# Autodesk Inventor assembly: Backpack
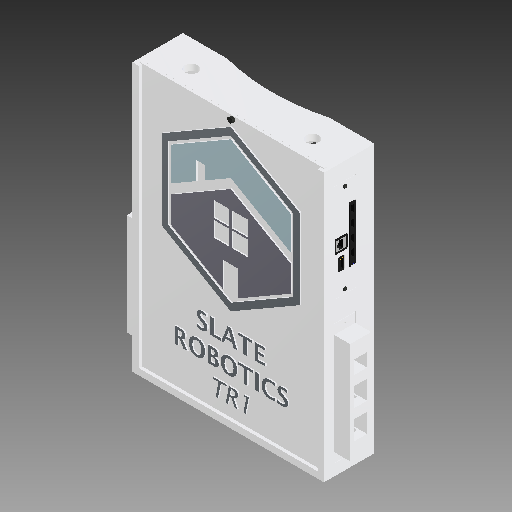
[picture p0: Inventor's stored thumbnail of the model, 512x512]
Saved by Autodesk Inventor 2017 (Build 210142000, 142)
## iProperties
Created: 2017-09-05
Part Number: Backpack
Document SubType Name: Assembly
Designer: Zach
Author: Zach
## Documents named in this file (18)
- C:\Users\Dell\Documents\GitHub\tr1\src\Body\Chest Assembly\Backpack Assembly\Backpack.iam
- C:\Users\Dell\Documents\GitHub\tr1\src\Body\Chest Assembly\Backpack Assembly\BP001b.ipt
- C:\Users\Dell\Documents\GitHub\tr1\src\Body\Chest Assembly\Backpack Assembly\BP002b.ipt
- C:\Users\Dell\Documents\GitHub\tr1\src\Body\Chest Assembly\Backpack Assembly\BP003.ipt
- C:\Users\Dell\Documents\GitHub\tr1\src\Body\Chest Assembly\Backpack Assembly\BP005.ipt
- C:\Users\Dell\Documents\GitHub\tr1\src\Body\Chest Assembly\Backpack Assembly\BP006.ipt
- C:\Users\Dell\Documents\GitHub\tr1\lib\Terminal Block 4\Клемная колодка ТВ-2504L 600V-25A\Клемная колодка ТВ-2504L 600V-25A.iam
- C:\Users\Dell\Documents\GitHub\tr1\lib\Arduino Mega 2560\Arduino Mega 2560.ipt
- C:\Users\Dell\Documents\GitHub\tr1\lib\L298n Driver\l298n.ipt
- C:\Users\Dell\Documents\GitHub\tr1\lib\Content Center Files\R2017\en-US\ISO 7045  H\ISO 7045 - M3 x 12 - 4.8 - H - ISO.ipt
- C:\Users\Dell\Documents\GitHub\tr1\lib\Content Center Files\R2017\en-US\ISO 4018\ISO 4018 - M5 x 25.ipt
- C:\Users\Dell\Documents\GitHub\tr1\src\Body\Chest Assembly\Backpack Assembly\USB Hub.ipt
- C:\Users\Dell\Documents\GitHub\tr1\src\Body\Chest Assembly\Backpack Assembly\HDMI Port.ipt
- C:\Users\Dell\Documents\GitHub\tr1\src\Body\Chest Assembly\Backpack Assembly\Ethernet Port.ipt
- C:\Users\Dell\Documents\GitHub\tr1\lib\Content Center Files\R2017\en-US\ISO 4035(2)\ISO 4035 - M3 - ISO.ipt
- C:\Users\Dell\Documents\GitHub\tr1\src\Body\Chest Assembly\Backpack Assembly\BP011.ipt
- C:\Users\Dell\Documents\GitHub\tr1\src\Body\Chest Assembly\Backpack Assembly\BP012.ipt
- C:\Users\Dell\Documents\GitHub\tr1\src\Body\Chest Assembly\Backpack Assembly\BP013.ipt
## Components (84 placed, 17 different names)
1. BP001b:1 — Mate:8, Mate:9, Mate:11, Mate:13, Mate:15, Mate:19, Mate:20, Mate:21, Mate:22, Mate:23, Flush:1, Mate:26, Mate:36, Mate:37, Mate:38, Mate:39, Mate:133, Mate:134, Mate:137, Mate:138, Mate:160, Mate:162, Mate:163, Mate:176, Mate:177, Mate:178, Mate:179, Mate:180, Mate:181, Mate:182, Mate:183, Mate:184, Mate:185, Mate:186, Mate:187, Mate:188, Mate:189, Mate:190, Mate:191, Mate:310, Mate:312, Mate:314, Mate:316, Mate:317, Mate:318, Mate:319, Mate:326, Mate:327, Mate:328, Mate:330, Mate:331, Mate:332, Mate:334, Mate:335, Mate:336, Mate:337, Mate:338, Mate:339, Mate:340, Mate:341, Mate:342, Mate:343, Mate:344, Mate:345, Mate:346, Mate:347, Mate:348, Mate:349, Mate:350, Mate:351
2. BP002b:1 — Mate:317, Mate:318, Mate:319, Mate:333
3. BP003:1 — Mate:15, Mate:36, Mate:37, Mate:65, Mate:66, Mate:67, Mate:68, Mate:69, Mate:70, Mate:135, Mate:136, Mate:232, Mate:233, Mate:234, Mate:235, Mate:236, Mate:237, Mate:238, Mate:239, Mate:240, Mate:241, Mate:242, Mate:243
4. BP003:2 — Mate:19, Mate:38, Mate:39, Mate:59, Mate:60, Mate:61, Mate:62, Mate:63, Mate:64, Mate:139, Mate:140, Mate:208, Mate:209, Mate:210, Mate:211, Mate:212, Mate:213, Mate:214, Mate:215, Mate:216, Mate:217, Mate:218, Mate:219
5. BP005:1 — Mate:8, Mate:9, Mate:20, Mate:172, Mate:173, Mate:174, Mate:175, Mate:307, Mate:308
6. BP006:1 — Mate:11, Mate:13, Mate:21, Mate:168, Mate:169, Mate:170, Mate:171, Flush:6, Mate:282, Mate:283, Flush:7, Mate:284, Mate:285, Flush:8, Mate:286
7. BP011:1 — Mate:342, Mate:343, Mate:344
8. BP012:1 — Mate:345, Mate:346, Mate:347
9. BP013:1 — Mate:348, Mate:349, Mate:351
10. Клемная колодка ТВ-2504L 600V-25A:1 [sub-assembly] — Mate:26, Mate:337, Mate:338
11. Клемная колодка ТВ-2504L 600V-25A:2 [sub-assembly] — Mate:339, Mate:340, Mate:341
12. Клемная колодка ТВ-2504L 600V-25A:3 [sub-assembly] — Mate:334, Mate:335, Mate:336
13. Arduino Mega 2560:1 — Mate:96, Mate:116, Mate:117, Mate:118, Mate:119, Mate:120, Mate:327, Mate:328, Mate:329
14. Arduino Mega 2560:2 — Mate:127, Mate:128, Mate:129, Mate:130, Mate:131, Mate:132, Mate:326, Mate:330, Mate:331
15. l298n:1 — Mate:59, Mate:60, Flush:3, Mate:228, Mate:229, Mate:230, Mate:231
16. l298n:2 — Mate:62, Mate:63, Flush:2, Flush:3, Mate:224, Mate:225, Mate:226, Mate:227
17. l298n:3 — Mate:61, Mate:64, Flush:2, Mate:220, Mate:221, Mate:222, Mate:223
18. l298n:4 — Mate:67, Mate:70, Flush:4, Flush:5, Mate:248, Mate:249, Mate:250, Mate:251
19. l298n:5 — Mate:68, Mate:69, Flush:5, Mate:252, Mate:253, Mate:254, Mate:255
20. l298n:6 — Mate:65, Mate:66, Flush:4, Mate:244, Mate:245, Mate:246, Mate:247
21. USB Hub:1 — Flush:6, Mate:286, Mate:350
22. HDMI Port:1 — Mate:282, Mate:283, Flush:7
23. Ethernet Port:1 — Mate:284, Mate:285, Flush:8
24. ISO 7045 H M3 x 12 - 4.8 - H:1 — Mate:96, Mate:329
25. ISO 7045 H M3 x 12 - 4.8 - H:2 — Mate:117
26. ISO 7045 H M3 x 12 - 4.8 - H:3 — Mate:119
27. ISO 7045 H M3 x 12 - 4.8 - H:4 — Mate:120
28. ISO 7045 H M3 x 12 - 4.8 - H:5 — Mate:118
29. ISO 7045 H M3 x 12 - 4.8 - H:6 — Mate:116
30. ISO 7045 H M3 x 12 - 4.8 - H:7 — Mate:128
31. ISO 7045 H M3 x 12 - 4.8 - H:8 — Mate:131
32. ISO 7045 H M3 x 12 - 4.8 - H:9 — Mate:132
33. ISO 7045 H M3 x 12 - 4.8 - H:10 — Mate:129
34. ISO 7045 H M3 x 12 - 4.8 - H:11 — Mate:130
35. ISO 7045 H M3 x 12 - 4.8 - H:12 — Mate:127
36. ISO 7045 H M3 x 12 - 4.8 - H:13 — Mate:133, Mate:136
37. ISO 7045 H M3 x 12 - 4.8 - H:14 — Mate:134, Mate:135
38. ISO 7045 H M3 x 12 - 4.8 - H:15 — Mate:137, Mate:139
39. ISO 7045 H M3 x 12 - 4.8 - H:16 — Mate:138, Mate:140
40. ISO 7045 H M3 x 12 - 4.8 - H:27 — Mate:160
41. ISO 7045 H M3 x 12 - 4.8 - H:28 — Mate:163
42. ISO 7045 H M3 x 12 - 4.8 - H:30 — Mate:162
43. ISO 7045 H M3 x 12 - 4.8 - H:31 — Mate:169, Mate:170, Mate:313
44. ISO 7045 H M3 x 12 - 4.8 - H:32 — Mate:168, Mate:171, Mate:315
45. ISO 7045 H M3 x 12 - 4.8 - H:33 — Mate:172, Mate:173, Mate:309
46. ISO 7045 H M3 x 12 - 4.8 - H:34 — Mate:174, Mate:175
47. ISO 4018 M5 x 25:5 — Mate:179, Mate:190
48. ISO 4018 M5 x 25:6 — Mate:181, Mate:186
49. ISO 4018 M5 x 25:7 — Mate:182, Mate:187
50. ISO 4018 M5 x 25:8 — Mate:180, Mate:189
51. ISO 4018 M5 x 25:9 — Mate:177, Mate:191
52. ISO 4018 M5 x 25:10 — Mate:176, Mate:184
53. ISO 4018 M5 x 25:11 — Mate:178, Mate:185
54. ISO 4018 M5 x 25:12 — Mate:183, Mate:188
55. ISO 7045 H M3 x 12 - 4.8 - H:35 — Mate:219, Mate:230
56. ISO 7045 H M3 x 12 - 4.8 - H:36 — Mate:218, Mate:229
57. ISO 7045 H M3 x 12 - 4.8 - H:37 — Mate:217, Mate:228
58. ISO 7045 H M3 x 12 - 4.8 - H:38 — Mate:215, Mate:225
59. ISO 7045 H M3 x 12 - 4.8 - H:39 — Mate:216, Mate:231
60. ISO 7045 H M3 x 12 - 4.8 - H:40 — Mate:214, Mate:224
61. ISO 7045 H M3 x 12 - 4.8 - H:41 — Mate:213, Mate:226
62. ISO 7045 H M3 x 12 - 4.8 - H:42 — Mate:211, Mate:222
63. ISO 7045 H M3 x 12 - 4.8 - H:43 — Mate:210, Mate:223
64. ISO 7045 H M3 x 12 - 4.8 - H:44 — Mate:212, Mate:227
65. ISO 7045 H M3 x 12 - 4.8 - H:45 — Mate:209, Mate:220
66. ISO 7045 H M3 x 12 - 4.8 - H:46 — Mate:208, Mate:221
67. ISO 7045 H M3 x 12 - 4.8 - H:47 — Mate:238, Mate:248
68. ISO 7045 H M3 x 12 - 4.8 - H:48 — Mate:239, Mate:250
69. ISO 7045 H M3 x 12 - 4.8 - H:49 — Mate:243, Mate:254
70. ISO 7045 H M3 x 12 - 4.8 - H:50 — Mate:242, Mate:255
71. ISO 7045 H M3 x 12 - 4.8 - H:51 — Mate:232, Mate:245
72. ISO 7045 H M3 x 12 - 4.8 - H:52 — Mate:233, Mate:244
73. ISO 7045 H M3 x 12 - 4.8 - H:53 — Mate:235, Mate:246
74. ISO 7045 H M3 x 12 - 4.8 - H:54 — Mate:234, Mate:247
75. ISO 7045 H M3 x 12 - 4.8 - H:55 — Mate:236, Mate:249
76. ISO 7045 H M3 x 12 - 4.8 - H:56 — Mate:237, Mate:251
77. ISO 7045 H M3 x 12 - 4.8 - H:57 — Mate:240, Mate:253
78. ISO 7045 H M3 x 12 - 4.8 - H:58 — Mate:241, Mate:252
79. ISO 7045 H M3 x 12 - 4.8 - H:67 — Mate:307, Mate:308, Mate:311
80. ISO 4035 M3:1 — Mate:309, Mate:310
81. ISO 4035 M3:2 — Mate:311, Mate:312
82. ISO 4035 M3:3 — Mate:313, Mate:314
83. ISO 4035 M3:4 — Mate:315, Mate:316
84. ISO 4018 M5 x 25:13 — Mate:332, Mate:333
## Relationships (174: Mate 166, Flush 8)
- Mate:8: BP001b:1 ↔ BP005:1
- Mate:9: BP001b:1 ↔ BP005:1
- Mate:11: BP001b:1 ↔ BP006:1
- Mate:13: BP001b:1 ↔ BP006:1
- Mate:15: BP001b:1 ↔ BP003:1
- Mate:19: BP001b:1 ↔ BP003:2
- Mate:20: BP001b:1 ↔ BP005:1
- Mate:21: BP001b:1 ↔ BP006:1
- Mate:22: BP001b:1
- Mate:23: BP001b:1
- Flush:1 (200 mm): BP001b:1
- Mate:26: BP001b:1 ↔ Клемная колодка ТВ-2504L 600V-25A:1
- Mate:36: BP001b:1 ↔ BP003:1
- Mate:37: BP001b:1 ↔ BP003:1
- Mate:38: BP001b:1 ↔ BP003:2
- Mate:39: BP001b:1 ↔ BP003:2
- Mate:59: BP003:2 ↔ l298n:1
- Mate:60: BP003:2 ↔ l298n:1
- Mate:61: BP003:2 ↔ l298n:3
- Mate:62: BP003:2 ↔ l298n:2
- Mate:63: BP003:2 ↔ l298n:2
- Mate:64: BP003:2 ↔ l298n:3
- Flush:2: l298n:2 ↔ l298n:3
- Flush:3: l298n:1 ↔ l298n:2
- Mate:65: BP003:1 ↔ l298n:6
- Mate:66: BP003:1 ↔ l298n:6
- Mate:67: BP003:1 ↔ l298n:4
- Mate:68: BP003:1 ↔ l298n:5
- Mate:69: BP003:1 ↔ l298n:5
- Mate:70: BP003:1 ↔ l298n:4
- Flush:4: l298n:4 ↔ l298n:6
- Flush:5: l298n:4 ↔ l298n:5
- Mate:96: Arduino Mega 2560:1 ↔ ISO 7045 H M3 x 12 - 4.8 - H:1
- Mate:116: Arduino Mega 2560:1 ↔ ISO 7045 H M3 x 12 - 4.8 - H:6
- Mate:117: Arduino Mega 2560:1 ↔ ISO 7045 H M3 x 12 - 4.8 - H:2
- Mate:118: Arduino Mega 2560:1 ↔ ISO 7045 H M3 x 12 - 4.8 - H:5
- Mate:119: Arduino Mega 2560:1 ↔ ISO 7045 H M3 x 12 - 4.8 - H:3
- Mate:120: Arduino Mega 2560:1 ↔ ISO 7045 H M3 x 12 - 4.8 - H:4
- Mate:127: Arduino Mega 2560:2 ↔ ISO 7045 H M3 x 12 - 4.8 - H:12
- Mate:128: Arduino Mega 2560:2 ↔ ISO 7045 H M3 x 12 - 4.8 - H:7
- Mate:129: Arduino Mega 2560:2 ↔ ISO 7045 H M3 x 12 - 4.8 - H:10
- Mate:130: Arduino Mega 2560:2 ↔ ISO 7045 H M3 x 12 - 4.8 - H:11
- Mate:131: Arduino Mega 2560:2 ↔ ISO 7045 H M3 x 12 - 4.8 - H:8
- Mate:132: Arduino Mega 2560:2 ↔ ISO 7045 H M3 x 12 - 4.8 - H:9
- Mate:133: BP001b:1 ↔ ISO 7045 H M3 x 12 - 4.8 - H:13
- Mate:134: BP001b:1 ↔ ISO 7045 H M3 x 12 - 4.8 - H:14
- Mate:135: BP003:1 ↔ ISO 7045 H M3 x 12 - 4.8 - H:14
- Mate:136: BP003:1 ↔ ISO 7045 H M3 x 12 - 4.8 - H:13
- Mate:137: BP001b:1 ↔ ISO 7045 H M3 x 12 - 4.8 - H:15
- Mate:138: BP001b:1 ↔ ISO 7045 H M3 x 12 - 4.8 - H:16
- Mate:139: BP003:2 ↔ ISO 7045 H M3 x 12 - 4.8 - H:15
- Mate:140: BP003:2 ↔ ISO 7045 H M3 x 12 - 4.8 - H:16
- Mate:160: BP001b:1 ↔ ISO 7045 H M3 x 12 - 4.8 - H:27
- Mate:162: BP001b:1 ↔ ISO 7045 H M3 x 12 - 4.8 - H:30
- Mate:163: BP001b:1 ↔ ISO 7045 H M3 x 12 - 4.8 - H:28
- Mate:168: BP006:1 ↔ ISO 7045 H M3 x 12 - 4.8 - H:32
- Mate:169: BP006:1 ↔ ISO 7045 H M3 x 12 - 4.8 - H:31
- Mate:170: BP006:1 ↔ ISO 7045 H M3 x 12 - 4.8 - H:31
- Mate:171: BP006:1 ↔ ISO 7045 H M3 x 12 - 4.8 - H:32
- Mate:172: BP005:1 ↔ ISO 7045 H M3 x 12 - 4.8 - H:33
- Mate:173: BP005:1 ↔ ISO 7045 H M3 x 12 - 4.8 - H:33
- Mate:174: BP005:1 ↔ ISO 7045 H M3 x 12 - 4.8 - H:34
- Mate:175: BP005:1 ↔ ISO 7045 H M3 x 12 - 4.8 - H:34
- Mate:176: BP001b:1 ↔ ISO 4018 M5 x 25:10
- Mate:177: BP001b:1 ↔ ISO 4018 M5 x 25:9
- Mate:178: BP001b:1 ↔ ISO 4018 M5 x 25:11
- Mate:179: BP001b:1 ↔ ISO 4018 M5 x 25:5
- Mate:180: BP001b:1 ↔ ISO 4018 M5 x 25:8
- Mate:181: BP001b:1 ↔ ISO 4018 M5 x 25:6
- Mate:182: BP001b:1 ↔ ISO 4018 M5 x 25:7
- Mate:183: BP001b:1 ↔ ISO 4018 M5 x 25:12
- Mate:184: BP001b:1 ↔ ISO 4018 M5 x 25:10
- Mate:185: BP001b:1 ↔ ISO 4018 M5 x 25:11
- Mate:186: BP001b:1 ↔ ISO 4018 M5 x 25:6
- Mate:187: BP001b:1 ↔ ISO 4018 M5 x 25:7
- Mate:188: BP001b:1 ↔ ISO 4018 M5 x 25:12
- Mate:189: BP001b:1 ↔ ISO 4018 M5 x 25:8
- Mate:190: BP001b:1 ↔ ISO 4018 M5 x 25:5
- Mate:191: BP001b:1 ↔ ISO 4018 M5 x 25:9
- Mate:208: BP003:2 ↔ ISO 7045 H M3 x 12 - 4.8 - H:46
- Mate:209: BP003:2 ↔ ISO 7045 H M3 x 12 - 4.8 - H:45
- Mate:210: BP003:2 ↔ ISO 7045 H M3 x 12 - 4.8 - H:43
- Mate:211: BP003:2 ↔ ISO 7045 H M3 x 12 - 4.8 - H:42
- Mate:212: BP003:2 ↔ ISO 7045 H M3 x 12 - 4.8 - H:44
- Mate:213: BP003:2 ↔ ISO 7045 H M3 x 12 - 4.8 - H:41
- Mate:214: BP003:2 ↔ ISO 7045 H M3 x 12 - 4.8 - H:40
- Mate:215: BP003:2 ↔ ISO 7045 H M3 x 12 - 4.8 - H:38
- Mate:216: BP003:2 ↔ ISO 7045 H M3 x 12 - 4.8 - H:39
- Mate:217: BP003:2 ↔ ISO 7045 H M3 x 12 - 4.8 - H:37
- Mate:218: BP003:2 ↔ ISO 7045 H M3 x 12 - 4.8 - H:36
- Mate:219: BP003:2 ↔ ISO 7045 H M3 x 12 - 4.8 - H:35
- Mate:220: l298n:3 ↔ ISO 7045 H M3 x 12 - 4.8 - H:45
- Mate:221: l298n:3 ↔ ISO 7045 H M3 x 12 - 4.8 - H:46
- Mate:222: l298n:3 ↔ ISO 7045 H M3 x 12 - 4.8 - H:42
- Mate:223: l298n:3 ↔ ISO 7045 H M3 x 12 - 4.8 - H:43
- Mate:224: l298n:2 ↔ ISO 7045 H M3 x 12 - 4.8 - H:40
- Mate:225: l298n:2 ↔ ISO 7045 H M3 x 12 - 4.8 - H:38
- Mate:226: l298n:2 ↔ ISO 7045 H M3 x 12 - 4.8 - H:41
- Mate:227: l298n:2 ↔ ISO 7045 H M3 x 12 - 4.8 - H:44
- Mate:228: l298n:1 ↔ ISO 7045 H M3 x 12 - 4.8 - H:37
- Mate:229: l298n:1 ↔ ISO 7045 H M3 x 12 - 4.8 - H:36
- Mate:230: l298n:1 ↔ ISO 7045 H M3 x 12 - 4.8 - H:35
- Mate:231: l298n:1 ↔ ISO 7045 H M3 x 12 - 4.8 - H:39
- Mate:232: BP003:1 ↔ ISO 7045 H M3 x 12 - 4.8 - H:51
- Mate:233: BP003:1 ↔ ISO 7045 H M3 x 12 - 4.8 - H:52
- Mate:234: BP003:1 ↔ ISO 7045 H M3 x 12 - 4.8 - H:54
- Mate:235: BP003:1 ↔ ISO 7045 H M3 x 12 - 4.8 - H:53
- Mate:236: BP003:1 ↔ ISO 7045 H M3 x 12 - 4.8 - H:55
- Mate:237: BP003:1 ↔ ISO 7045 H M3 x 12 - 4.8 - H:56
- Mate:238: BP003:1 ↔ ISO 7045 H M3 x 12 - 4.8 - H:47
- Mate:239: BP003:1 ↔ ISO 7045 H M3 x 12 - 4.8 - H:48
- Mate:240: BP003:1 ↔ ISO 7045 H M3 x 12 - 4.8 - H:57
- Mate:241: BP003:1 ↔ ISO 7045 H M3 x 12 - 4.8 - H:58
- Mate:242: BP003:1 ↔ ISO 7045 H M3 x 12 - 4.8 - H:50
- Mate:243: BP003:1 ↔ ISO 7045 H M3 x 12 - 4.8 - H:49
- Mate:244: l298n:6 ↔ ISO 7045 H M3 x 12 - 4.8 - H:52
- Mate:245: l298n:6 ↔ ISO 7045 H M3 x 12 - 4.8 - H:51
- Mate:246: l298n:6 ↔ ISO 7045 H M3 x 12 - 4.8 - H:53
- Mate:247: l298n:6 ↔ ISO 7045 H M3 x 12 - 4.8 - H:54
- Mate:248: l298n:4 ↔ ISO 7045 H M3 x 12 - 4.8 - H:47
- Mate:249: l298n:4 ↔ ISO 7045 H M3 x 12 - 4.8 - H:55
- Mate:250: l298n:4 ↔ ISO 7045 H M3 x 12 - 4.8 - H:48
- Mate:251: l298n:4 ↔ ISO 7045 H M3 x 12 - 4.8 - H:56
- Mate:252: l298n:5 ↔ ISO 7045 H M3 x 12 - 4.8 - H:58
- Mate:253: l298n:5 ↔ ISO 7045 H M3 x 12 - 4.8 - H:57
- Mate:254: l298n:5 ↔ ISO 7045 H M3 x 12 - 4.8 - H:49
- Mate:255: l298n:5 ↔ ISO 7045 H M3 x 12 - 4.8 - H:50
- Flush:6: BP006:1 ↔ USB Hub:1
- Mate:282 (0.5 mm): BP006:1 ↔ HDMI Port:1
- Mate:283 (0.5 mm): BP006:1 ↔ HDMI Port:1
- Flush:7: BP006:1 ↔ HDMI Port:1
- Mate:284: BP006:1 ↔ Ethernet Port:1
- Mate:285 (0.5 mm): BP006:1 ↔ Ethernet Port:1
- Flush:8: BP006:1 ↔ Ethernet Port:1
- Mate:286 (0.5 mm): BP006:1 ↔ USB Hub:1
- Mate:307: BP005:1 ↔ ISO 7045 H M3 x 12 - 4.8 - H:67
- Mate:308: BP005:1 ↔ ISO 7045 H M3 x 12 - 4.8 - H:67
- Mate:309: ISO 7045 H M3 x 12 - 4.8 - H:33 ↔ ISO 4035 M3:1
- Mate:310: BP001b:1 ↔ ISO 4035 M3:1
- Mate:311: ISO 7045 H M3 x 12 - 4.8 - H:67 ↔ ISO 4035 M3:2
- Mate:312: BP001b:1 ↔ ISO 4035 M3:2
- Mate:313: ISO 7045 H M3 x 12 - 4.8 - H:31 ↔ ISO 4035 M3:3
- Mate:314: BP001b:1 ↔ ISO 4035 M3:3
- Mate:315: ISO 7045 H M3 x 12 - 4.8 - H:32 ↔ ISO 4035 M3:4
- Mate:316: BP001b:1 ↔ ISO 4035 M3:4
- Mate:317: BP001b:1 ↔ BP002b:1
- Mate:318 (1 mm): BP001b:1 ↔ BP002b:1
- Mate:319: BP001b:1 ↔ BP002b:1
- Mate:326: BP001b:1 ↔ Arduino Mega 2560:2
- Mate:327: BP001b:1 ↔ Arduino Mega 2560:1
- Mate:328: BP001b:1 ↔ Arduino Mega 2560:1
- Mate:329: Arduino Mega 2560:1 ↔ ISO 7045 H M3 x 12 - 4.8 - H:1
- Mate:330: BP001b:1 ↔ Arduino Mega 2560:2
- Mate:331: BP001b:1 ↔ Arduino Mega 2560:2
- Mate:332: BP001b:1 ↔ ISO 4018 M5 x 25:13
- Mate:333: BP002b:1 ↔ ISO 4018 M5 x 25:13
- Mate:334: BP001b:1 ↔ Клемная колодка ТВ-2504L 600V-25A:3
- Mate:335: BP001b:1 ↔ Клемная колодка ТВ-2504L 600V-25A:3
- Mate:336: BP001b:1 ↔ Клемная колодка ТВ-2504L 600V-25A:3
- Mate:337: BP001b:1 ↔ Клемная колодка ТВ-2504L 600V-25A:1
- Mate:338: BP001b:1 ↔ Клемная колодка ТВ-2504L 600V-25A:1
- Mate:339: BP001b:1 ↔ Клемная колодка ТВ-2504L 600V-25A:2
- Mate:340: BP001b:1 ↔ Клемная колодка ТВ-2504L 600V-25A:2
- Mate:341: BP001b:1 ↔ Клемная колодка ТВ-2504L 600V-25A:2
- Mate:342: BP001b:1 ↔ BP011:1
- Mate:343: BP001b:1 ↔ BP011:1
- Mate:344: BP001b:1 ↔ BP011:1
- Mate:345: BP001b:1 ↔ BP012:1
- Mate:346: BP001b:1 ↔ BP012:1
- Mate:347: BP001b:1 ↔ BP012:1
- Mate:348: BP001b:1 ↔ BP013:1
- Mate:349: BP001b:1 ↔ BP013:1
- Mate:350: BP001b:1 ↔ USB Hub:1
- Mate:351: BP001b:1 ↔ BP013:1
